# Autodesk Inventor assembly: full guns 2
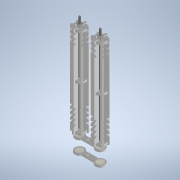
[picture p0: Inventor's stored thumbnail of the model, 180x180]
Saved by Autodesk Inventor 2020.1 (Build 241239000, 239)
## iProperties
Created: 2022-03-19
Part Number: full guns 2
Document SubType Name: Assembly
Designer: User
Author: User
## Documents named in this file (4)
- D:\GitHub\TANK\3D-turret\full guns 2.iam
- D:\GitHub\TANK\3D-turret\gun.iam
- D:\GitHub\TANK\3D-turret\соединение пушек.ipt
- D:\GitHub\TANK\3D-turret\подшипник.ipt
## Components (8 placed, 3 different names)
1. gun:2 [sub-assembly]
2. gun:3 [sub-assembly]
3. соединение пушек:2
4. подшипник:3
5. подшипник:4
6. соединение пушек:3
7. подшипник:5
8. подшипник:6
## Relationships (4: WeldJoint 4)
- [WeldJoint]: соединение пушек:2 ↔ подшипник:3
- [WeldJoint]: соединение пушек:2 ↔ подшипник:4
- [WeldJoint]: соединение пушек:3 ↔ подшипник:5
- [WeldJoint]: соединение пушек:3 ↔ подшипник:6
## Named parameters: d10_d0 = 0 mm, d11_d1 = 0 mm, d15_d0 = 0 mm, d16_d1 = 0 mm
